# Autodesk Inventor assembly: 20X20lift
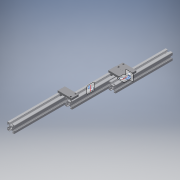
[picture p0: Inventor's stored thumbnail of the model, 180x180]
Saved by Autodesk Inventor 2017 (Build 210142000, 142)
## iProperties
Created: 2017-12-15
Part Number: 20X20lift
Document SubType Name: Assembly
Designer: User
Author: User
## Documents named in this file (3)
- C:\Robotics\CAD\2017-18_CAD\20X20lift.iam
- C:\Robotics\CAD\2017-18_CAD\Prototypes\Sliderfor2020.ipt
- C:\Robotics\CAD\COTSParts\Bosch Extrusion\Bosch 20x20 6 in.ipt
## Components (6 placed, 2 different names)
1. Sliderfor2020:1 — Mate:1, Mate:2, Flush:6
2. Bosch 20x20 6 in:1 — Mate:1, Mate:2, Mate:3, Flush:1, Flush:3, Mate:4, Flush:4, Flush:5
3. Bosch 20x20 6 in:2 — Mate:3, Flush:1, Mate:7, Mate:8, Flush:6
4. Bosch 20x20 6 in:3 — Flush:3, Mate:4, Mate:5, Mate:6
5. Sliderfor2020:2 — Mate:7, Mate:8, Flush:5
6. Sliderfor2020:3 — Mate:5, Mate:6, Flush:4
## Relationships (13: Mate 8, Flush 5)
- Mate:1: Sliderfor2020:1 ↔ Bosch 20x20 6 in:1
- Mate:2 (0.6223 mm): Sliderfor2020:1 ↔ Bosch 20x20 6 in:1
- Mate:3 (1 mm): Bosch 20x20 6 in:1 ↔ Bosch 20x20 6 in:2
- Flush:1: Bosch 20x20 6 in:1 ↔ Bosch 20x20 6 in:2
- Flush:3: Bosch 20x20 6 in:1 ↔ Bosch 20x20 6 in:3
- Mate:4 (1 mm): Bosch 20x20 6 in:1 ↔ Bosch 20x20 6 in:3
- Mate:5: Bosch 20x20 6 in:3 ↔ Sliderfor2020:3
- Mate:6 (0.6223 mm): Bosch 20x20 6 in:3 ↔ Sliderfor2020:3
- Flush:4: Bosch 20x20 6 in:1 ↔ Sliderfor2020:3
- Mate:7: Bosch 20x20 6 in:2 ↔ Sliderfor2020:2
- Mate:8 (0.6223 mm): Bosch 20x20 6 in:2 ↔ Sliderfor2020:2
- Flush:5: Bosch 20x20 6 in:1 ↔ Sliderfor2020:2
- Flush:6 (114.3 mm): Sliderfor2020:1 ↔ Bosch 20x20 6 in:2
